# Autodesk Inventor assembly: P1699_EG
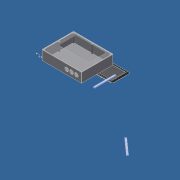
[picture p0: Inventor's stored thumbnail of the model, 180x180]
Saved by Autodesk Inventor 2015 SP2 (Build 190223200, 223)
## iProperties
Created: 2017-06-14
Part Number: P1699_EG
Project: Nom Projet
Description: Ens. Nom Ensemble
Document SubType Name: Assembly
Designer: Francis-Lucien-Hugue
Author: Francis-Lucien-Hugue
## Documents named in this file (7)
- C:\Users\Francis-Lucien-Hugue\Desktop\TimbreuseLocal\hardware\box\P1699_EG.iam
- C:\Users\Francis-Lucien-Hugue\Desktop\TimbreuseLocal\hardware\box\Box.ipt
- C:\Users\Francis-Lucien-Hugue\Desktop\TimbreuseLocal\hardware\box\P1699_002_FaceAvant.ipt
- C:\Users\Francis-Lucien-Hugue\Desktop\TimbreuseLocal\hardware\box\Imported Components\Raspberry_Pi_Touch_Screen_Assembly_-_Pins_Out\Raspberry_Pi_Touch_Screen_Assembly_-_Pins_Out.iam
- C:\Users\Francis-Lucien-Hugue\Desktop\TimbreuseLocal\hardware\box\P1699_003_Support.ipt
- C:\Users\Francis-Lucien-Hugue\Documents\Inventor\Content Center Files\R2015\fr-FR\DIN 912\DIN 912 - M3 x 0.5 x 8 x 6.75.ipt
- C:\Users\Francis-Lucien-Hugue\Documents\Inventor\Content Center Files\R2015\fr-FR\DIN 912\DIN 912 - M3 x 0.5 x 12 x 10.75.ipt
## Components (13 placed, 5 different names)
1. Box:1 — Placage:1, Placage:2, Placage:3
2. Pièce1:1 — Placage:1, Placage:2, Placage:3
3. Raspberry_Pi_Touch_Screen_Assembly_-_Pins_Out:1 [sub-assembly]
4. Pièce1:2
5. Pièce1:3
6. DIN 912 - Remplacé par DIN EN ISO 4762 M3 x 8:1
7. DIN 912 - Remplacé par DIN EN ISO 4762 M3 x 8:2
8. DIN 912 - Remplacé par DIN EN ISO 4762 M3 x 8:3
9. DIN 912 - Remplacé par DIN EN ISO 4762 M3 x 8:4
10. DIN 912 - Remplacé par DIN EN ISO 4762 M3 x 12:1
11. DIN 912 - Remplacé par DIN EN ISO 4762 M3 x 12:2
12. DIN 912 - Remplacé par DIN EN ISO 4762 M3 x 12:3
13. DIN 912 - Remplacé par DIN EN ISO 4762 M3 x 12:4
## Relationships (3: Mate 3)
- Placage:1 [Mate]: Box:1 ↔ Pièce1:1
- Placage:2 [Mate]: Box:1 ↔ Pièce1:1
- Placage:3 [Mate]: Box:1 ↔ Pièce1:1
